# Autodesk Inventor assembly: DPLX_A003_Lab_Version_Small_RevB
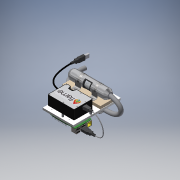
[picture p0: Inventor's stored thumbnail of the model, 180x180]
Saved by Autodesk Inventor 2018 (Build 220112000, 112)
## iProperties
Created: 2018-06-12
Part Number: DPLX_A003_Lab_Version_Small_RevB
Document SubType Name: Assembly
Designer: DPLXuser
Author: DPLXuser
## Documents named in this file (18)
- C:\Users\DPLXuser\Documents\Michael Schwab\SPARK CAD Files\DPLX_A003_Lab_Version_Small_RevB.iam
- C:\Users\DPLXuser\Documents\Michael Schwab\SPARK CAD Files\DPLX_P014_Lab_Baseplate_Small_PV.ipt
- C:\Users\DPLXuser\Documents\Michael Schwab\SPARK CAD Files\DPLX_P017_.5in _Standoff_smallplate.ipt
- C:\Users\DPLXuser\Documents\wire_t_to_b.ipt
- C:\Users\DPLXuser\Documents\Michael Schwab\SPARK CAD Files\DPLX_P021_Standoff_Rasp_pie_Lab_payload_sv.ipt
- C:\Users\DPLXuser\Documents\Michael Schwab\SPARK CAD Files\DPLX_A004_VIPE_Lab.iam
- C:\Users\DPLXuser\Documents\Michael Schwab\SPARK CAD Files\DPLX_P024_Ocean Optics Flame.iam
- C:\Users\DPLXuser\Documents\Michael Schwab\SPARK CAD Files\DPLX_A005_Spark_Gap_Lab.iam
- C:\Users\DPLXuser\Documents\Michael Schwab\SPARK CAD Files\DPLX_A006_RPi3.iam
- C:\Users\DPLXuser\Documents\Michael Schwab\SPARK CAD Files\91828A211_TYPE 18-8 STAINLESS STEEL HEX NUT.ipt
- C:\Users\DPLXuser\Documents\Michael Schwab\SPARK CAD Files\DPLX_P036 mini USB.ipt
- C:\Users\DPLXuser\Documents\Michael Schwab\SPARK CAD Files\DPLX_P037 USB.ipt
- C:\Users\DPLXuser\Documents\Michael Schwab\SPARK CAD Files\usb Wire.ipt
- C:\Users\DPLXuser\Documents\Michael Schwab\SPARK CAD Files\Wire to Spark Gap.ipt
- C:\Users\DPLXuser\Documents\Michael Schwab\SPARK CAD Files\Wire to Power.ipt
- C:\Users\DPLXuser\Documents\Michael Schwab\SPARK CAD Files\DPLX_P038 Micro USB.ipt
- C:\Users\DPLXuser\Documents\Michael Schwab\SPARK CAD Files\Pi Wire.ipt
- C:\Users\DPLXuser\Documents\Michael Schwab\SPARK CAD Files\91771A085_18-8 SS FLAT HEAD PHILLIPS MACHINE SCREW 2-56 .875in.ipt
## Components (36 placed, 17 different names)
1. DPLX_P014_Lab_Baseplate_Small_PV:1 — Insert:1, Insert:2, Mate:23, Insert:34, Insert:35, Insert:36, Insert:37, Insert:51, Insert:52, Insert:53, Insert:54, Insert:55, Insert:56, Insert:58, Insert:60, Mate:24, Insert:63, Insert:64, Insert:65, Insert:66, Insert:67, Insert:68, Insert:69, Insert:70, Insert:74, Insert:75, Insert:76
2. DPLX_P017_.5in _Standoff_smallplate:2 — Insert:2, Insert:59
3. DPLX_P017_.5in _Standoff_smallplate:3 — Insert:1, Insert:57, Insert:58
4. DPLX_P017_.5in _Standoff_smallplate:4 — Mate:23
5. wire_t_to_b:1 — Flush:11, Flush:12
6. DPLX_P021_Standoff_Rasp_pie_Lab_payload_sv:1 — Insert:34, Insert:62
7. DPLX_P021_Standoff_Rasp_pie_Lab_payload_sv:2 — Insert:36
8. DPLX_P021_Standoff_Rasp_pie_Lab_payload_sv:3 — Insert:37
9. DPLX_P021_Standoff_Rasp_pie_Lab_payload_sv:4 — Insert:35, Insert:61
10. DPLX_P021_Standoff_Rasp_pie_Lab_payload_sv:5 — Insert:54
11. DPLX_P021_Standoff_Rasp_pie_Lab_payload_sv:6 — Insert:52
12. DPLX_P021_Standoff_Rasp_pie_Lab_payload_sv:7 — Insert:51
13. DPLX_P021_Standoff_Rasp_pie_Lab_payload_sv:8 — Insert:53
14. DPLX_A004_VIPE_Lab:1 [sub-assembly] — Insert:55, Insert:56, Insert:72
15. DPLX_P024_Ocean Optics Flame:1 [sub-assembly] — Insert:57, Insert:59, Insert:71
16. DPLX_A005_Spark_Gap_Lab:1 [sub-assembly] — Insert:60, Mate:24, Flush:16
17. DPLX_A006_RPi3:1 [sub-assembly] — Insert:61, Insert:62, Mate:25, Mate:27, Mate:28, Mate:30
18. 91828A211_TYPE 18-8 STAINLESS STEEL HEX NUT:1 — Insert:68
19. 91828A211_TYPE 18-8 STAINLESS STEEL HEX NUT:2 — Insert:70
20. 91828A211_TYPE 18-8 STAINLESS STEEL HEX NUT:3 — Insert:69
21. 91828A211_TYPE 18-8 STAINLESS STEEL HEX NUT:4 — Insert:66
22. 91828A211_TYPE 18-8 STAINLESS STEEL HEX NUT:5 — Insert:63
23. 91828A211_TYPE 18-8 STAINLESS STEEL HEX NUT:6 — Insert:67
24. 91828A211_TYPE 18-8 STAINLESS STEEL HEX NUT:7 — Insert:64
25. 91828A211_TYPE 18-8 STAINLESS STEEL HEX NUT:8 — Insert:65
26. DPLX_P036 mini USB:1 — Insert:71, Flush:13, Mate:26
27. DPLX_P037 USB:1 — Mate:25, Flush:14
28. usb Wire:1 — Flush:13, Flush:14, Mate:26
29. Wire to Spark Gap:1 — Flush:15, Flush:16
30. Wire to Power:1 — Insert:72, Mate:29
31. DPLX_P038 Micro USB:1 — Mate:27, Mate:28, Flush:17
32. Pi Wire:1 — Flush:17, Mate:29, Mate:30, Insert:73
33. DPLX_P037 USB:2 — Insert:73
34. 91771A085_18-8 SS FLAT HEAD PHILLIPS MACHINE SCREW 2-56 .875in:1 — Insert:74
35. 91771A085_18-8 SS FLAT HEAD PHILLIPS MACHINE SCREW 2-56 .875in:2 — Insert:76
36. 91771A085_18-8 SS FLAT HEAD PHILLIPS MACHINE SCREW 2-56 .875in:3 — Insert:75
## Relationships (47: Insert 32, Mate 8, Flush 7)
- Insert:1: DPLX_P014_Lab_Baseplate_Small_PV:1 ↔ DPLX_P017_.5in _Standoff_smallplate:3
- Insert:2: DPLX_P014_Lab_Baseplate_Small_PV:1 ↔ DPLX_P017_.5in _Standoff_smallplate:2
- Mate:23: DPLX_P014_Lab_Baseplate_Small_PV:1 ↔ DPLX_P017_.5in _Standoff_smallplate:4
- Flush:11: wire_t_to_b:1
- Flush:12: wire_t_to_b:1
- Insert:34: DPLX_P014_Lab_Baseplate_Small_PV:1 ↔ DPLX_P021_Standoff_Rasp_pie_Lab_payload_sv:1
- Insert:35: DPLX_P014_Lab_Baseplate_Small_PV:1 ↔ DPLX_P021_Standoff_Rasp_pie_Lab_payload_sv:4
- Insert:36: DPLX_P014_Lab_Baseplate_Small_PV:1 ↔ DPLX_P021_Standoff_Rasp_pie_Lab_payload_sv:2
- Insert:37: DPLX_P014_Lab_Baseplate_Small_PV:1 ↔ DPLX_P021_Standoff_Rasp_pie_Lab_payload_sv:3
- Insert:51: DPLX_P014_Lab_Baseplate_Small_PV:1 ↔ DPLX_P021_Standoff_Rasp_pie_Lab_payload_sv:7
- Insert:52: DPLX_P014_Lab_Baseplate_Small_PV:1 ↔ DPLX_P021_Standoff_Rasp_pie_Lab_payload_sv:6
- Insert:53: DPLX_P014_Lab_Baseplate_Small_PV:1 ↔ DPLX_P021_Standoff_Rasp_pie_Lab_payload_sv:8
- Insert:54: DPLX_P014_Lab_Baseplate_Small_PV:1 ↔ DPLX_P021_Standoff_Rasp_pie_Lab_payload_sv:5
- Insert:55: DPLX_P014_Lab_Baseplate_Small_PV:1 ↔ DPLX_A004_VIPE_Lab:1
- Insert:56: DPLX_P014_Lab_Baseplate_Small_PV:1 ↔ DPLX_A004_VIPE_Lab:1
- Insert:57: DPLX_P017_.5in _Standoff_smallplate:3 ↔ DPLX_P024_Ocean Optics Flame:1
- Insert:58: DPLX_P014_Lab_Baseplate_Small_PV:1 ↔ DPLX_P017_.5in _Standoff_smallplate:3
- Insert:59: DPLX_P017_.5in _Standoff_smallplate:2 ↔ DPLX_P024_Ocean Optics Flame:1
- Insert:60: DPLX_P014_Lab_Baseplate_Small_PV:1 ↔ DPLX_A005_Spark_Gap_Lab:1
- Mate:24: DPLX_P014_Lab_Baseplate_Small_PV:1 ↔ DPLX_A005_Spark_Gap_Lab:1
- Insert:61: DPLX_P021_Standoff_Rasp_pie_Lab_payload_sv:4 ↔ DPLX_A006_RPi3:1
- Insert:62: DPLX_P021_Standoff_Rasp_pie_Lab_payload_sv:1 ↔ DPLX_A006_RPi3:1
- Insert:63: DPLX_P014_Lab_Baseplate_Small_PV:1 ↔ 91828A211_TYPE 18-8 STAINLESS STEEL HEX NUT:5
- Insert:64: DPLX_P014_Lab_Baseplate_Small_PV:1 ↔ 91828A211_TYPE 18-8 STAINLESS STEEL HEX NUT:7
- Insert:65: DPLX_P014_Lab_Baseplate_Small_PV:1 ↔ 91828A211_TYPE 18-8 STAINLESS STEEL HEX NUT:8
- Insert:66: DPLX_P014_Lab_Baseplate_Small_PV:1 ↔ 91828A211_TYPE 18-8 STAINLESS STEEL HEX NUT:4
- Insert:67: DPLX_P014_Lab_Baseplate_Small_PV:1 ↔ 91828A211_TYPE 18-8 STAINLESS STEEL HEX NUT:6
- Insert:68: DPLX_P014_Lab_Baseplate_Small_PV:1 ↔ 91828A211_TYPE 18-8 STAINLESS STEEL HEX NUT:1
- Insert:69: DPLX_P014_Lab_Baseplate_Small_PV:1 ↔ 91828A211_TYPE 18-8 STAINLESS STEEL HEX NUT:3
- Insert:70: DPLX_P014_Lab_Baseplate_Small_PV:1 ↔ 91828A211_TYPE 18-8 STAINLESS STEEL HEX NUT:2
- Insert:71 (-7.62 mm): DPLX_P024_Ocean Optics Flame:1 ↔ DPLX_P036 mini USB:1
- Mate:25: DPLX_A006_RPi3:1 ↔ DPLX_P037 USB:1
- Flush:13: DPLX_P036 mini USB:1 ↔ usb Wire:1
- Flush:14: DPLX_P037 USB:1 ↔ usb Wire:1
- Mate:26: DPLX_P036 mini USB:1 ↔ usb Wire:1
- Flush:15: Wire to Spark Gap:1
- Flush:16: DPLX_A005_Spark_Gap_Lab:1 ↔ Wire to Spark Gap:1
- Insert:72: DPLX_A004_VIPE_Lab:1 ↔ Wire to Power:1
- Mate:27: DPLX_A006_RPi3:1 ↔ DPLX_P038 Micro USB:1
- Mate:28: DPLX_A006_RPi3:1 ↔ DPLX_P038 Micro USB:1
- Flush:17: DPLX_P038 Micro USB:1 ↔ Pi Wire:1
- Mate:29: Wire to Power:1 ↔ Pi Wire:1
- Mate:30: DPLX_A006_RPi3:1 ↔ Pi Wire:1
- Insert:73: Pi Wire:1 ↔ DPLX_P037 USB:2
- Insert:74: DPLX_P014_Lab_Baseplate_Small_PV:1 ↔ 91771A085_18-8 SS FLAT HEAD PHILLIPS MACHINE SCREW 2-56 .875in:1
- Insert:75: DPLX_P014_Lab_Baseplate_Small_PV:1 ↔ 91771A085_18-8 SS FLAT HEAD PHILLIPS MACHINE SCREW 2-56 .875in:3
- Insert:76: DPLX_P014_Lab_Baseplate_Small_PV:1 ↔ 91771A085_18-8 SS FLAT HEAD PHILLIPS MACHINE SCREW 2-56 .875in:2
